# Autodesk Inventor assembly: R1_version0
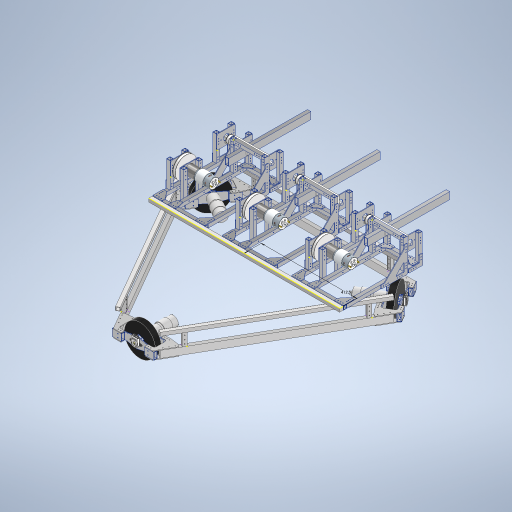
[picture p0: Inventor's stored thumbnail of the model, 512x512]
Saved by Autodesk Inventor 2023 (Build 270158000, 158)
## iProperties
Created: 2022-04-26
Part Number: R1_version0
Document SubType Name: Assembly
Designer: yuta
Author: yuta
## Documents named in this file (4)
- C:\Users\yuta\Documents\NHK\R1_version0.iam
- C:\Users\yuta\Documents\NHK\足回り.iam
- C:\Users\yuta\Documents\NHK\射出機構.iam
- C:\Users\yuta\Documents\NHK\試作_825.ipt
## Components (5 placed, 3 different names)
1. 足回り:1 [sub-assembly] — メイト:3, メイト:4, メイト:5
2. 射出機構:1 [sub-assembly] — メイト:1, フラッシュ:1, フラッシュ:2
3. 射出機構:2 [sub-assembly] — メイト:1, フラッシュ:1, フラッシュ:2, メイト:2, フラッシュ:3, フラッシュ:4
4. 射出機構:3 [sub-assembly] — メイト:2, フラッシュ:3, フラッシュ:4, メイト:6
5. 試作_825:1 — メイト:3, メイト:4, メイト:5, メイト:6
## Relationships (10: Mate 6, Flush 4)
- メイト:1 [Mate] (285 mm): 射出機構:1 ↔ 射出機構:2
- フラッシュ:1 [Flush]: 射出機構:1 ↔ 射出機構:2
- フラッシュ:2 [Flush]: 射出機構:1 ↔ 射出機構:2
- メイト:2 [Mate] (285 mm): 射出機構:2 ↔ 射出機構:3
- フラッシュ:3 [Flush]: 射出機構:2 ↔ 射出機構:3
- フラッシュ:4 [Flush]: 射出機構:2 ↔ 射出機構:3
- メイト:3 [Mate]: 足回り:1 ↔ 試作_825:1
- メイト:4 [Mate]: 足回り:1 ↔ 試作_825:1
- メイト:5 [Mate] (-345 mm): 足回り:1 ↔ 試作_825:1
- メイト:6 [Mate]: 射出機構:3 ↔ 試作_825:1
